# Autodesk Inventor assembly: Piston Subassembly
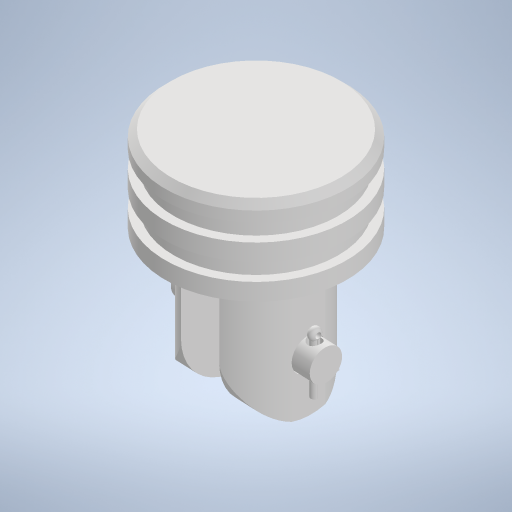
[picture p0: Inventor's stored thumbnail of the model, 512x512]
Saved by Autodesk Inventor 2023 (Build 270158000, 158)
## iProperties
Created: 2022-12-22
Part Number: Piston Subassembly
Document SubType Name: Assembly
Designer: tgr41
Author: tgr41
## Documents named in this file (4)
- C:\Users\tgr41\OneDrive\Documents\Repositories\3D-Prints\Steam Engine 2 Inch V3\Piston Subassembly.iam
- C:\Users\tgr41\OneDrive\Documents\Repositories\Steam-Engine\2 Inch V3\Piston 2.ipt
- C:\Users\tgr41\OneDrive\Documents\Repositories\Steam-Engine\2 Inch V3\Wrist Pin.ipt
- C:\Users\tgr41\OneDrive\Documents\Repositories\Steam-Engine\2 Inch V3\Cotter Pin.ipt
## Components (4 placed, 3 different names)
1. Piston 2:1 — Mate:1, Tangent:2, Angle:1, Angle:2, Angle:3, Angle:4
2. Wrist Pin:1 — Mate:1, Mate:2, Tangent:1, Tangent:2, Mate:3, Tangent:3
3. Cotter Pin:1 — Mate:3, Tangent:3, Angle:2, Angle:4
4. Cotter Pin:2 — Mate:2, Tangent:1, Angle:1, Angle:3
## Relationships (10: Angle 4, Mate 3, Tangent 3)
- Mate:1: Piston 2:1 ↔ Wrist Pin:1
- Mate:2: Wrist Pin:1 ↔ Cotter Pin:2
- Tangent:1: Wrist Pin:1 ↔ Cotter Pin:2
- Tangent:2: Piston 2:1 ↔ Wrist Pin:1
- Angle:1 (90 deg): Piston 2:1 ↔ Cotter Pin:2
- Mate:3: Wrist Pin:1 ↔ Cotter Pin:1
- Tangent:3: Wrist Pin:1 ↔ Cotter Pin:1
- Angle:2 (-90 deg): Piston 2:1 ↔ Cotter Pin:1
- Angle:3 (180 deg): Piston 2:1 ↔ Cotter Pin:2
- Angle:4 (0 deg): Piston 2:1 ↔ Cotter Pin:1
